# Autodesk Inventor assembly: Ensamblaje1
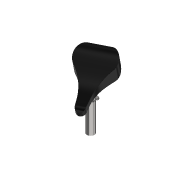
[picture p0: Inventor's stored thumbnail of the model, 180x180]
Saved by Autodesk Inventor 2021 (Build 250183000, 183)
## iProperties
Created: 2013-06-06
Part Number: Ensamblaje1
Document SubType Name: Assembly
Designer: BRAYAN
Author: BRAYAN
## Documents named in this file (9)
- C:\Users\maaro\Documents\UNAL\Automatización de Procesos de Manufactura\Github\Proyecto_APM\02 Inventor\sillin.iam
- C:\Users\maaro\Documents\UNAL\Automatización de Procesos de Manufactura\Github\Proyecto_APM\02 Inventor\Partes Sillín\tubo_sillin.ipt
- C:\Users\maaro\Documents\UNAL\Automatización de Procesos de Manufactura\Github\Proyecto_APM\02 Inventor\Partes Sillín\tuerca_sillin.ipt
- C:\Users\maaro\Documents\UNAL\Automatización de Procesos de Manufactura\Github\Proyecto_APM\02 Inventor\Partes Sillín\agarre_sillin.ipt
- C:\Users\maaro\Documents\UNAL\Automatización de Procesos de Manufactura\Github\Proyecto_APM\02 Inventor\Partes Sillín\tornillo_sillin.ipt
- C:\Users\maaro\Documents\UNAL\Automatización de Procesos de Manufactura\Github\Proyecto_APM\02 Inventor\Partes Sillín\ajuste_varilla_principal.ipt
- C:\Users\maaro\Documents\UNAL\Automatización de Procesos de Manufactura\Github\Proyecto_APM\02 Inventor\Partes Sillín\ajuste_varilla_secundario.ipt
- C:\Users\maaro\Documents\UNAL\Automatización de Procesos de Manufactura\Github\Proyecto_APM\02 Inventor\Partes Sillín\varilla_sillin.ipt
- C:\Users\maaro\Documents\UNAL\Automatización de Procesos de Manufactura\Github\Proyecto_APM\02 Inventor\Partes Sillín\sillin.ipt
## Components (11 placed, 8 different names)
1. tubo_sillin:1 — Insertar:1
2. agarre_sillin:1 — Insertar:1, Insertar:2, Insertar:3, Insertar:4, Coincidencia:1
3. tornillo_sillin:1 — Insertar:4, Insertar:5, Insertar:6, Insertar:7, Insertar:8
4. tuerca_sillin:2 — Insertar:7
5. tuerca_sillin:1 — Insertar:8
6. ajuste_varilla_principal:1 — Insertar:2, Coincidencia:2, Insert:9
7. ajuste_varilla_principal:2 — Insertar:3, Coincidencia:1, Coincidencia:2, Coincidencia:4, Coincidencia:5
8. ajuste_varilla_secundario:1 — Insertar:5, Coincidencia:3
9. ajuste_varilla_secundario:2 — Insertar:6, Coincidencia:3, Coincidencia:4
10. varilla_sillin:1 — Insert:9, Coincidencia:5, Insertar:10, Coincidencia:6
11. sillin:1 — Insertar:10, Coincidencia:6
## Relationships (16: Insert 10, Mate 6)
- Insertar:1: tubo_sillin:1 ↔ agarre_sillin:1
- Insertar:2 (-3.5 mm): agarre_sillin:1 ↔ ajuste_varilla_principal:1
- Insertar:3 (2 mm): agarre_sillin:1 ↔ ajuste_varilla_principal:2
- Insertar:4 (-8 mm): agarre_sillin:1 ↔ tornillo_sillin:1
- Insertar:5 (6 mm): tornillo_sillin:1 ↔ ajuste_varilla_secundario:1
- Insertar:6 (6 mm): tornillo_sillin:1 ↔ ajuste_varilla_secundario:2
- Insertar:7 (-3.8 mm): tornillo_sillin:1 ↔ tuerca_sillin:2
- Insertar:8 (-3.8 mm): tornillo_sillin:1 ↔ tuerca_sillin:1
- Coincidencia:1 [Mate]: agarre_sillin:1 ↔ ajuste_varilla_principal:2
- Coincidencia:2 [Mate]: ajuste_varilla_principal:1 ↔ ajuste_varilla_principal:2
- Coincidencia:3 [Mate]: ajuste_varilla_secundario:1 ↔ ajuste_varilla_secundario:2
- Coincidencia:4 [Mate]: ajuste_varilla_principal:2 ↔ ajuste_varilla_secundario:2
- Insert:9 (-50 mm): ajuste_varilla_principal:1 ↔ varilla_sillin:1
- Coincidencia:5 [Mate]: ajuste_varilla_principal:2 ↔ varilla_sillin:1
- Insertar:10 (-10 mm): varilla_sillin:1 ↔ sillin:1
- Coincidencia:6 [Mate]: varilla_sillin:1 ↔ sillin:1
